# Autodesk Inventor assembly: Sheathing_For_Side
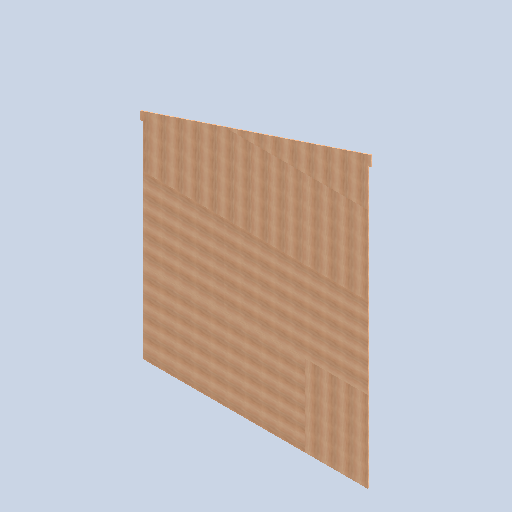
[picture p0: Inventor's stored thumbnail of the model, 512x512]
Saved by Autodesk Inventor 2025 (Build 290162010, 162A)
## iProperties
Created: 2024-10-03
Part Number: Sheathing_For_Side
Document SubType Name: Assembly
Designer: Tom
Author: Tom
## Documents named in this file (8)
- C:\Users\Tom\Documents\Inventor\Mobility\Additional_Building\Sheathing_For_Side.iam
- C:\Users\Tom\Documents\Inventor\Mobility\Additional_Building\OSB_For_Walls_With_Dimensions_48_x_96_Inches.ipt
- C:\Users\Tom\Documents\Inventor\Mobility\Additional_Building\OSB_For_Walls_With_Dimensions_37_x_48_Inches.ipt
- C:\Users\Tom\Documents\Inventor\Mobility\Additional_Building\OSB_For_Walls_With_Dimensions_48_x_48_Inches.ipt
- C:\Users\Tom\Documents\Inventor\Mobility\Additional_Building\OSB_For_Walls_With_Dimensions_48_x_85_Inches.ipt
- C:\Users\Tom\Documents\Inventor\Mobility\Additional_Building\OSB_For_Side_And_Back.ipt
- C:\Users\Tom\Documents\Inventor\Mobility\Additional_Building\OSB_For_Side_And_Front.ipt
- C:\Users\Tom\Documents\Inventor\Mobility\Additional_Building\OSB_For_Side_And_Top.ipt
## Components (7 placed, 7 different names)
1. OSB_For_Walls_With_Dimensions_48_x_96_Inches:1 — Mate:1, Mate:2, Mate:3, Mate:4, Flush:1, Flush:2, Mate:5, Flush:3, Flush:4, Flush:11, Flush:12, Flush:13
2. OSB_For_Walls_With_Dimensions_37_x_48_Inches:1 — Mate:4, Flush:1, Flush:2, Mate:6, Flush:13, Flush:14
3. OSB_For_Walls_With_Dimensions_48_x_48_Inches:1 — Mate:5, Flush:3, Flush:4, Mate:7, Mate:8, Flush:5, Flush:6, Flush:11, Flush:15, Flush:16
4. OSB_For_Walls_With_Dimensions_48_x_85_Inches:1 — Mate:6, Mate:7, Mate:9, Flush:7, Flush:8, Flush:12, Flush:14, Flush:15, Flush:17
5. OSB_For_Side_And_Back:1 — Mate:8, Flush:5, Flush:6, Flush:16, Flush:18
6. OSB_For_Side_And_Front:1 — Mate:9, Flush:7, Flush:8, Mate:10, Flush:9, Flush:10, Flush:17, Flush:19
7. OSB_For_Side_And_Top:1 — Mate:10, Flush:9, Flush:10, Flush:18, Flush:19
## Relationships (29: Flush 19, Mate 10)
- Mate:1: OSB_For_Walls_With_Dimensions_48_x_96_Inches:1
- Mate:2: OSB_For_Walls_With_Dimensions_48_x_96_Inches:1
- Mate:3: OSB_For_Walls_With_Dimensions_48_x_96_Inches:1
- Mate:4: OSB_For_Walls_With_Dimensions_48_x_96_Inches:1 ↔ OSB_For_Walls_With_Dimensions_37_x_48_Inches:1
- Flush:1: OSB_For_Walls_With_Dimensions_48_x_96_Inches:1 ↔ OSB_For_Walls_With_Dimensions_37_x_48_Inches:1
- Flush:2: OSB_For_Walls_With_Dimensions_48_x_96_Inches:1 ↔ OSB_For_Walls_With_Dimensions_37_x_48_Inches:1
- Mate:5: OSB_For_Walls_With_Dimensions_48_x_96_Inches:1 ↔ OSB_For_Walls_With_Dimensions_48_x_48_Inches:1
- Flush:3: OSB_For_Walls_With_Dimensions_48_x_96_Inches:1 ↔ OSB_For_Walls_With_Dimensions_48_x_48_Inches:1
- Flush:4: OSB_For_Walls_With_Dimensions_48_x_96_Inches:1 ↔ OSB_For_Walls_With_Dimensions_48_x_48_Inches:1
- Mate:6: OSB_For_Walls_With_Dimensions_37_x_48_Inches:1 ↔ OSB_For_Walls_With_Dimensions_48_x_85_Inches:1
- Mate:7: OSB_For_Walls_With_Dimensions_48_x_48_Inches:1 ↔ OSB_For_Walls_With_Dimensions_48_x_85_Inches:1
- Mate:8: OSB_For_Walls_With_Dimensions_48_x_48_Inches:1 ↔ OSB_For_Side_And_Back:1
- Flush:5: OSB_For_Walls_With_Dimensions_48_x_48_Inches:1 ↔ OSB_For_Side_And_Back:1
- Flush:6: OSB_For_Walls_With_Dimensions_48_x_48_Inches:1 ↔ OSB_For_Side_And_Back:1
- Mate:9: OSB_For_Walls_With_Dimensions_48_x_85_Inches:1 ↔ OSB_For_Side_And_Front:1
- Flush:7: OSB_For_Walls_With_Dimensions_48_x_85_Inches:1 ↔ OSB_For_Side_And_Front:1
- Flush:8: OSB_For_Walls_With_Dimensions_48_x_85_Inches:1 ↔ OSB_For_Side_And_Front:1
- Mate:10: OSB_For_Side_And_Front:1 ↔ OSB_For_Side_And_Top:1
- Flush:9: OSB_For_Side_And_Front:1 ↔ OSB_For_Side_And_Top:1
- Flush:10: OSB_For_Side_And_Front:1 ↔ OSB_For_Side_And_Top:1
- Flush:11: OSB_For_Walls_With_Dimensions_48_x_96_Inches:1 ↔ OSB_For_Walls_With_Dimensions_48_x_48_Inches:1
- Flush:12: OSB_For_Walls_With_Dimensions_48_x_96_Inches:1 ↔ OSB_For_Walls_With_Dimensions_48_x_85_Inches:1
- Flush:13: OSB_For_Walls_With_Dimensions_48_x_96_Inches:1 ↔ OSB_For_Walls_With_Dimensions_37_x_48_Inches:1
- Flush:14: OSB_For_Walls_With_Dimensions_37_x_48_Inches:1 ↔ OSB_For_Walls_With_Dimensions_48_x_85_Inches:1
- Flush:15: OSB_For_Walls_With_Dimensions_48_x_48_Inches:1 ↔ OSB_For_Walls_With_Dimensions_48_x_85_Inches:1
- Flush:16: OSB_For_Walls_With_Dimensions_48_x_48_Inches:1 ↔ OSB_For_Side_And_Back:1
- Flush:17: OSB_For_Walls_With_Dimensions_48_x_85_Inches:1 ↔ OSB_For_Side_And_Front:1
- Flush:18: OSB_For_Side_And_Back:1 ↔ OSB_For_Side_And_Top:1
- Flush:19: OSB_For_Side_And_Front:1 ↔ OSB_For_Side_And_Top:1
